# Autodesk Inventor assembly: Packing
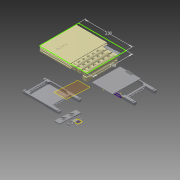
[picture p0: Inventor's stored thumbnail of the model, 180x180]
Saved by Autodesk Inventor 2015 (Build 190159000, 159)
## iProperties
Created: 2015-04-21
Part Number: Packing
Document SubType Name: Assembly
Designer: Akovo_000
Author: Akovo_000
## Documents named in this file (11)
- C:\Users\Akovo_000\SkyDrive\3D printing\Enclosure Half-Open\Packing.iam
- C:\Users\Akovo_000\SkyDrive\3D printing\Enclosure Half-Open\SidePanelNarrow.ipt
- C:\Users\Akovo_000\SkyDrive\3D printing\Enclosure Half-Open\SidePanelNarrowWithPowerButton.ipt
- C:\Users\Akovo_000\SkyDrive\3D printing\Enclosure Half-Open\SidePanelwide.ipt
- C:\Users\Akovo_000\SkyDrive\3D printing\Enclosure Half-Open\Pillar.ipt
- C:\Users\Akovo_000\SkyDrive\3D printing\Enclosure Half-Open\NUCholder.ipt
- C:\Users\Akovo_000\SkyDrive\3D printing\Enclosure Half-Open\Lid_clip.ipt
- C:\Users\Akovo_000\SkyDrive\3D printing\Enclosure Half-Open\Lid.ipt
- C:\Users\Akovo_000\SkyDrive\3D printing\Enclosure Half-Open\LensPlane.ipt
- C:\Users\Akovo_000\SkyDrive\3D printing\Enclosure Half-Open\GenericPanel.ipt
- C:\Users\Akovo_000\SkyDrive\3D printing\Enclosure Half-Open\FilterHolder.ipt
## Components (14 placed, 10 different names)
1. SidePanelNarrow:1
2. SidePanelNarrowWithPowerButton:1
3. SidePanelwide:1
4. SidePanelwide:2
5. Pillar:1
6. Pillar:2
7. Pillar:3
8. Pillar:4
9. NUCholder:1
10. Lid_clip:1
11. Lid:1
12. LensPlane:1
13. GenericPanel:1
14. FilterHolder:1 — Flush:1
## Relationships (1: Flush 1)
- Flush:1: FilterHolder:1
